# Autodesk Inventor assembly: genius invention 1
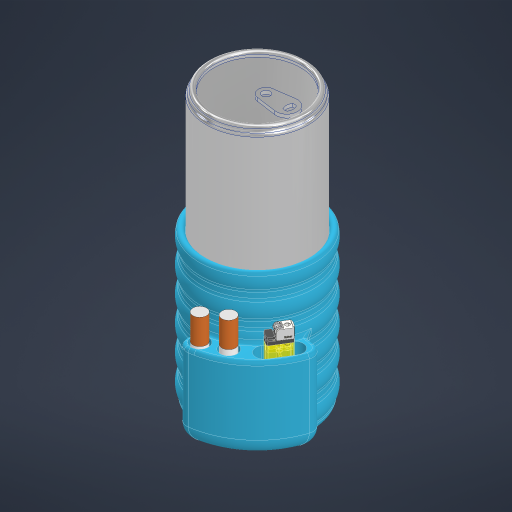
[picture p0: Inventor's stored thumbnail of the model, 512x512]
Saved by Autodesk Inventor 2024 (Build 280153000, 153)
## iProperties
Created: 2025-01-28
Part Number: genius invention 1
Document SubType Name: Assembly
Designer: turbo
Author: turbo
## Documents named in this file (5)
- C:\Shared\alex-bartella-schoolwork\4b03\genius invention 1.iam
- C:\Shared\alex-bartella-schoolwork\4b03\the cup.ipt
- C:\Shared\alex-bartella-schoolwork\4b03\icantputitdown.ipt
- C:\Shared\alex-bartella-schoolwork\4b03\Lighter.ipt
- C:\Shared\alex-bartella-schoolwork\4b03\ciggy.iam
## Components (5 placed, 4 different names)
1. the cup:1 — Mate:1, Mate:2
2. icantputitdown:1 — Mate:1, Mate:2, Mate:3, Mate:4, Mate:5
3. Lighter:1 — Mate:3
4. ciggy:1 [sub-assembly] — Mate:4
5. ciggy:2 [sub-assembly] — Mate:5
## Relationships (5: Mate 5)
- Mate:1: the cup:1 ↔ icantputitdown:1
- Mate:2: the cup:1 ↔ icantputitdown:1
- Mate:3 (2 mm): icantputitdown:1 ↔ Lighter:1
- Mate:4: icantputitdown:1 ↔ ciggy:1
- Mate:5: icantputitdown:1 ↔ ciggy:2
